# Autodesk Inventor assembly: Bridge
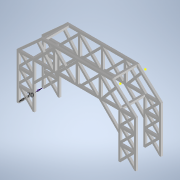
[picture p0: Inventor's stored thumbnail of the model, 180x180]
Saved by Autodesk Inventor 2020.1 (Build 241239000, 239)
## iProperties
Created: 2020-02-13
Part Number: Bridge
Document SubType Name: Assembly
Designer: super
Author: super
## Documents named in this file (14)
- C:\Users\super\Desktop\Giovanni\Science\3D Models\Autodesk-Inventor\Projects\Bridge\Bridge.iam
- C:\Users\super\Desktop\Giovanni\Science\3D Models\Autodesk-Inventor\Projects\Bridge\Longest.ipt
- C:\Users\super\Desktop\Giovanni\Science\3D Models\Autodesk-Inventor\Projects\Bridge\2ndFloorLongAngle.ipt
- C:\Users\super\Desktop\Giovanni\Science\3D Models\Autodesk-Inventor\Projects\Bridge\Bottom support.ipt
- C:\Users\super\Desktop\Giovanni\Science\3D Models\Autodesk-Inventor\Projects\Bridge\Angles in little squares.ipt
- C:\Users\super\Desktop\Giovanni\Science\3D Models\Autodesk-Inventor\Projects\Bridge\LittleConnection.ipt
- C:\Users\super\Desktop\Giovanni\Science\3D Models\Autodesk-Inventor\Projects\Bridge\Bottom support_MIR.ipt
- C:\Users\super\Desktop\Giovanni\Science\3D Models\Autodesk-Inventor\Projects\Bridge\Angles in little squares_MIR.ipt
- C:\Users\super\Desktop\Giovanni\Science\3D Models\Autodesk-Inventor\Projects\Bridge\LittleConnection_MIR.ipt
- C:\Users\super\Desktop\Giovanni\Science\3D Models\Autodesk-Inventor\Projects\Bridge\TopTop.ipt
- C:\Users\super\Desktop\Giovanni\Science\3D Models\Autodesk-Inventor\Projects\Bridge\MainAngle.ipt
- C:\Users\super\Desktop\Giovanni\Science\3D Models\Autodesk-Inventor\Projects\Bridge\2ndFloorSupport.ipt
- C:\Users\super\Desktop\Giovanni\Science\3D Models\Autodesk-Inventor\Projects\Bridge\2ndFloorOAngle.ipt
- C:\Users\super\Desktop\Giovanni\Science\3D Models\Autodesk-Inventor\Projects\Bridge\Connector.ipt
## Components (78 placed, 13 different names)
1. Longest:1 — Mate:1, Flush:1, Mate:2, Flush:2, Mate:3, Mate:4, Flush:5, Flush:6, Mate:11, Mate:12, Flush:9
2. 2ndFloorLongAngle:1 — Mate:2, Flush:2
3. 2ndFloorLongAngle:2 — Mate:1, Flush:1
4. Bottom support:1 — Mate:3, Flush:5, Mate:7
5. Bottom support:2 — Mate:4, Flush:6, Mate:8, Flush:7, Mate:13, Flush:10
6. Angles in little squares:1 — Mate:7
7. LittleConnection:1
8. Angles in little squares:2
9. LittleConnection:2
10. Angles in little squares:3
11. Angles in little squares:4 — Mate:8, Flush:7
12. Angles in little squares:5
13. Angles in little squares:6
14. Bottom support_MIR:1 — Mate:9
15. Bottom support_MIR:2 — Flush:8, Mate:10, Mate:14, Flush:11
16. Angles in little squares_MIR:1 — Mate:9
17. LittleConnection_MIR:1
18. Angles in little squares_MIR:2
19. LittleConnection_MIR:2
20. Angles in little squares_MIR:3
21. Angles in little squares_MIR:4 — Flush:8, Mate:10
22. Angles in little squares_MIR:5
23. Angles in little squares_MIR:6
24. TopTop:1
25. MainAngle:1 — Mate:11
26. MainAngle:2 — Mate:12, Flush:9
27. 2ndFloorSupport:1
28. 2ndFloorSupport:2
29. MainAngle:3 — Mate:13, Flush:10
30. MainAngle:4 — Mate:14, Flush:11
31. MainAngle:5
32. MainAngle:6
33. 2ndFloorSupport:3
34. MainAngle:7
35. MainAngle:8
36. 2ndFloorOAngle:1
37. 2ndFloorOAngle:2
38. Longest:2
39. 2ndFloorLongAngle:3
40. 2ndFloorLongAngle:4
41. Bottom support:3
42. Bottom support:4
43. Angles in little squares:7
44. LittleConnection:3
45. Angles in little squares:8
46. LittleConnection:4
47. Angles in little squares:9
48. Angles in little squares:10
49. Angles in little squares:11
50. Angles in little squares:12
51. Bottom support_MIR:3
52. Bottom support_MIR:4
53. Angles in little squares_MIR:7
54. LittleConnection_MIR:3
55. Angles in little squares_MIR:8
56. LittleConnection_MIR:4
57. Angles in little squares_MIR:9
58. Angles in little squares_MIR:10
59. Angles in little squares_MIR:11
60. Angles in little squares_MIR:12
61. TopTop:2
62. MainAngle:9
63. MainAngle:10
64. 2ndFloorSupport:4
65. 2ndFloorSupport:5
66. MainAngle:11
67. MainAngle:12
68. MainAngle:13
69. MainAngle:14
70. 2ndFloorSupport:6
71. MainAngle:15
72. MainAngle:16
73. 2ndFloorOAngle:3
74. 2ndFloorOAngle:4
75. Connector:1
76. Connector:2
77. Connector:3
78. Connector:4
## Relationships (42: Mate 24, Flush 18)
- Mate:1: Longest:1 ↔ 2ndFloorLongAngle:2
- Flush:1: Longest:1 ↔ 2ndFloorLongAngle:2
- Mate:2: Longest:1 ↔ 2ndFloorLongAngle:1
- Flush:2: Longest:1 ↔ 2ndFloorLongAngle:1
- Mate:3: Longest:1 ↔ Bottom support:1
- Mate:4: Longest:1 ↔ Bottom support:2
- Flush:5: Longest:1 ↔ Bottom support:1
- Flush:6: Longest:1 ↔ Bottom support:2
- Mate:7: Bottom support:1 ↔ Angles in little squares:1
- Mate:8: Bottom support:2 ↔ Angles in little squares:4
- Flush:7: Bottom support:2 ↔ Angles in little squares:4
- Mate:9: Bottom support_MIR:1 ↔ Angles in little squares_MIR:1
- Flush:8: Bottom support_MIR:2 ↔ Angles in little squares_MIR:4
- Mate:10: Bottom support_MIR:2 ↔ Angles in little squares_MIR:4
- Mate:11: Longest:1 ↔ MainAngle:1
- Mate:12: Longest:1 ↔ MainAngle:2
- Flush:9: Longest:1 ↔ MainAngle:2
- Mate:13: Bottom support:2 ↔ MainAngle:3
- Flush:10: Bottom support:2 ↔ MainAngle:3
- Mate:14: Bottom support_MIR:2 ↔ MainAngle:4
- Flush:11: Bottom support_MIR:2 ↔ MainAngle:4
- [Mate]: Longest:2 ↔ 2ndFloorLongAngle:4
- [Flush]: Longest:2 ↔ 2ndFloorLongAngle:4
- [Mate]: Longest:2 ↔ 2ndFloorLongAngle:3
- [Flush]: Longest:2 ↔ 2ndFloorLongAngle:3
- [Mate]: Longest:2 ↔ Bottom support:3
- [Mate]: Longest:2 ↔ Bottom support:4
- [Flush]: Longest:2 ↔ Bottom support:3
- [Flush]: Longest:2 ↔ Bottom support:4
- [Mate]: Bottom support:3 ↔ Angles in little squares:7
- [Mate]: Bottom support:4 ↔ Angles in little squares:10
- [Flush]: Bottom support:4 ↔ Angles in little squares:10
- [Mate]: Bottom support_MIR:3 ↔ Angles in little squares_MIR:7
- [Flush]: Bottom support_MIR:4 ↔ Angles in little squares_MIR:10
- [Mate]: Bottom support_MIR:4 ↔ Angles in little squares_MIR:10
- [Mate]: Longest:2 ↔ MainAngle:9
- [Mate]: Longest:2 ↔ MainAngle:10
- [Flush]: Longest:2 ↔ MainAngle:10
- [Mate]: Bottom support:4 ↔ MainAngle:11
- [Flush]: Bottom support:4 ↔ MainAngle:11
- [Mate]: Bottom support_MIR:4 ↔ MainAngle:12
- [Flush]: Bottom support_MIR:4 ↔ MainAngle:12
## Named parameters: d26_d0 = 0 mm, d27_d1 = 0 mm, d28_d2 = 0 mm, d29_d3 = 0 mm, d30_d4 = 0 mm, d31_d5 = 0 mm, d32_d10 = 0 mm, d33_d11 = 0 mm, d34_d12 = 0 mm, d35_d13 = 0 mm, d36_d14 = 0 mm, d37_d15 = 0 mm, d38_d16 = 0 mm, d39_d17 = 0 mm, d40_d18 = 0 mm, d41_d19 = 0 mm, d42_d20 = 0 mm, d43_d21 = 0 mm, d44_d22 = 0 mm, d45_d23 = 0 mm, d46_d24 = 0 mm
